# Autodesk Inventor assembly: WheelAssembly3.0
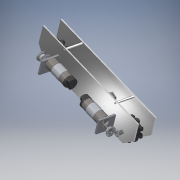
[picture p0: Inventor's stored thumbnail of the model, 180x180]
Saved by Autodesk Inventor 2019 (Build 230136000, 136)
## iProperties
Created: 2017-07-22
Part Number: WheelAssembly3.0
Document SubType Name: Assembly
Designer: User
Mass: 2301.48 g
Surface Area: 4071.67 cm^2
Volume: 902.346 cm^3
Density: 2.55055 g/cm^3
Author: User
## Documents named in this file (23)
- C:\Robotics\CAD\2020-21-CAD\Drivetrain\drive train left.iam
- C:\Robotics\CAD\2016-17_CAD\Custom COTS\4inax.ipt
- C:\Robotics\CAD\COTSParts\Actobotics\535 parts\535198Bearing.25ID.5OD.ipt
- C:\Robotics\CAD\COTSParts\Actobotics\Collar.ipt
- C:\Robotics\CAD\COTSParts\Fasteners\6-32 SHCS x500.ipt
- C:\Robotics\CAD\COTSParts\Fasteners\Hex Standoff 6-32 x2250.ipt
- C:\Robotics\CAD\COTSParts\Motors\am-3102NeveRest20 (1)_MIR.ipt
- C:\Robotics\CAD\COTSParts\Rev\REV-41-1657MecanumWheelRight.iam
- C:\Robotics\CAD\2020-21-CAD\Drivetrain\motor mount.ipt
- C:\Robotics\CAD\COTSParts\Tetrix\Tetrix hub - motor.ipt
- C:\Robotics\CAD\2016-17_CAD\Custom COTS\4inax_MIR1.ipt
- C:\Robotics\CAD\COTSParts\Actobotics\535 parts\535198Bearing.25ID.5OD_MIR1.ipt
- C:\Robotics\CAD\COTSParts\Actobotics\Collar_MIR1.ipt
- C:\Robotics\CAD\COTSParts\Rev\REV-41-1657MecanumWheelRight_MIR.iam
- C:\Robotics\CAD\2020-21-CAD\Drivetrain\motor mount_MIR.ipt
- C:\Robotics\CAD\COTSParts\Motors\am-3102NeveRest20 (1)_MIR_MIR.ipt
- C:\Robotics\CAD\COTSParts\andymark\am-3902 am-3903 2in Omni 14mm Hex.ipt
- C:\Robotics\CAD\COTSParts\Rev\REV-11-1271.STEP encoders.ipt
- C:\Robotics\CAD\COTSParts\Actobotics\637 parts\637222 beval gear\615456 13tooth beval gear.ipt
- C:\Robotics\CAD\COTSParts\Actobotics\637 parts\637222 beval gear\615460 26 tooth beval gear.ipt
- C:\Robotics\CAD\COTSParts\Tetrix\Tetrix Hub - axle.ipt
- C:\Robotics\CAD\2020-21-CAD\Drivetrain\InvertedDrivePlateOutsideright.ipt
- C:\Robotics\CAD\2020-21-CAD\Drivetrain\InvertedDrivePlateInsideleft.ipt
## Components (37 placed, 22 different names)
1. 4inax:4 — Mate:63, Mate:69, Mate:118, Mate:144, Mate:168, Mate:170
2. 535198Bearing.25ID.5OD:1 — Mate:116, Mate:145, Mate:171
3. Collar:1 — Mate:168, Mate:169
4. 535198Bearing.25ID.5OD:5 — Mate:117, Mate:118, Mate:169
5. Hex Standoff 6-32 x2250:1 — Mate:138, Mate:139
6. Hex Standoff 6-32 x2250:2 — Mate:114, Mate:130
7. Hex Standoff 6-32 x2250:3 — Mate:136, Mate:137
8. Hex Standoff 6-32 x2250:4 — Mate:140, Mate:141, Mate:146
9. 6-32 SHCS x500:22 — Mate:119, Mate:149
10. 6-32 SHCS x500:23 — Mate:124, Mate:125, Mate:141
11. 6-32 SHCS x500:24 — Mate:128, Mate:134, Mate:139
12. 6-32 SHCS x500:25 — Mate:129, Mate:130, Mate:131
13. 6-32 SHCS x500:26 — Mate:147, Mate:148
14. 6-32 SHCS x500:27 — Mate:132, Mate:135, Mate:137
15. 6-32 SHCS x500:28 — Mate:154, Mate:157
16. 6-32 SHCS x500:29 — Mate:155, Mate:156
17. REV-41-1657MecanumWheelRight:1 [sub-assembly] — Mate:63, Mate:70, Mate:71, Mate:72, Flush:14
18. motor mount:1 — Mate:66, Mate:67, Mate:113, Flush:16, Flush:20, Mate:162
19. am-3102NeveRest20 (1)_MIR:2 — Mate:66, Mate:67, Mate:112, Angle:8
20. Tetrix hub - motor:1 — Mate:69, Mate:70, Mate:71, Mate:72
21. 4inax_MIR1:1 — Mate:76, Mate:150, Mate:167, Mate:172, Mate:175
22. 535198Bearing.25ID.5OD_MIR1:1 — Mate:151, Mate:174
23. Collar_MIR1:1 — Mate:172, Mate:173
24. 535198Bearing.25ID.5OD_MIR1:2 — Mate:142, Mate:143, Mate:167, Mate:173
25. REV-41-1657MecanumWheelRight_MIR:1 [sub-assembly] — Mate:76, Flush:14, Mate:152
26. motor mount_MIR:1 — Angle:7, Mate:163, Flush:21, Flush:22, Mate:164, Mate:165, Mate:166
27. am-3102NeveRest20 (1)_MIR_MIR:1 — Mate:96, Angle:7, Mate:164, Mate:165, Angle:8
28. am-3902 am-3903 2in Omni 14mm Hex:1 — Mate:89, Mate:90
29. REV-11-1271.STEP encoders:1 — Mate:89, Mate:90, Mate:126, Mate:127, Angle:3
30. 615456 13tooth beval gear:1 — Mate:174, Mate:175
31. 615460 26 tooth beval gear:1 — Mate:93, Mate:94, Mate:96
32. Tetrix Hub - axle:1 — Mate:93, Mate:94, Mate:166
33. 615456 13tooth beval gear:2 — Mate:170, Mate:171
34. 615460 26 tooth beval gear:3 — Mate:113
35. Tetrix Hub - axle:3 — Mate:112
36. InvertedDrivePlateOutsideright:1 — Mate:114, Mate:116, Mate:117, Mate:119, Mate:124, Mate:125, Mate:126, Mate:127, Angle:3, Mate:128, Mate:129, Mate:131, Mate:132, Mate:134, Mate:135, Mate:136, Mate:138, Mate:140, Mate:142, Mate:143, Angle:4, Flush:16, Flush:20
37. InvertedDrivePlateInsideleft:1 — Mate:144, Mate:145, Mate:146, Angle:4, Mate:147, Mate:148, Mate:149, Mate:150, Mate:151, Mate:152, Mate:154, Mate:155, Mate:156, Mate:157, Mate:162, Mate:163, Flush:21, Flush:22
## Relationships (77: Mate 68, Flush 5, Angle 4)
- Mate:63: 4inax:4 ↔ REV-41-1657MecanumWheelRight:1
- Mate:66: motor mount:1 ↔ am-3102NeveRest20 (1)_MIR:2
- Mate:67: motor mount:1 ↔ am-3102NeveRest20 (1)_MIR:2
- Mate:69: 4inax:4 ↔ Tetrix hub - motor:1
- Mate:70: REV-41-1657MecanumWheelRight:1 ↔ Tetrix hub - motor:1
- Mate:71: REV-41-1657MecanumWheelRight:1 ↔ Tetrix hub - motor:1
- Mate:72: REV-41-1657MecanumWheelRight:1 ↔ Tetrix hub - motor:1
- Mate:76: 4inax_MIR1:1 ↔ REV-41-1657MecanumWheelRight_MIR:1
- Flush:14: REV-41-1657MecanumWheelRight:1 ↔ REV-41-1657MecanumWheelRight_MIR:1
- Mate:89: am-3902 am-3903 2in Omni 14mm Hex:1 ↔ REV-11-1271.STEP encoders:1
- Mate:90: am-3902 am-3903 2in Omni 14mm Hex:1 ↔ REV-11-1271.STEP encoders:1
- Mate:93: 615460 26 tooth beval gear:1 ↔ Tetrix Hub - axle:1
- Mate:94: 615460 26 tooth beval gear:1 ↔ Tetrix Hub - axle:1
- Mate:96: am-3102NeveRest20 (1)_MIR_MIR:1 ↔ 615460 26 tooth beval gear:1
- [Mate]: 615460 26 tooth beval gear:3 ↔ Tetrix Hub - axle:3
- [Mate]: 615460 26 tooth beval gear:3 ↔ Tetrix Hub - axle:3
- Mate:112: am-3102NeveRest20 (1)_MIR:2 ↔ Tetrix Hub - axle:3
- Mate:113 (25.4 mm): motor mount:1 ↔ 615460 26 tooth beval gear:3
- Mate:114: Hex Standoff 6-32 x2250:2 ↔ InvertedDrivePlateOutsideright:1
- Mate:116: 535198Bearing.25ID.5OD:1 ↔ InvertedDrivePlateOutsideright:1
- Mate:117: 535198Bearing.25ID.5OD:5 ↔ InvertedDrivePlateOutsideright:1
- Mate:118: 4inax:4 ↔ 535198Bearing.25ID.5OD:5
- Mate:119: 6-32 SHCS x500:22 ↔ InvertedDrivePlateOutsideright:1
- Mate:124: 6-32 SHCS x500:23 ↔ InvertedDrivePlateOutsideright:1
- Mate:125: 6-32 SHCS x500:23 ↔ InvertedDrivePlateOutsideright:1
- Mate:126: REV-11-1271.STEP encoders:1 ↔ InvertedDrivePlateOutsideright:1
- Mate:127: REV-11-1271.STEP encoders:1 ↔ InvertedDrivePlateOutsideright:1
- Angle:3 (25.25 deg): REV-11-1271.STEP encoders:1 ↔ InvertedDrivePlateOutsideright:1
- Mate:128: 6-32 SHCS x500:24 ↔ InvertedDrivePlateOutsideright:1
- Mate:129: 6-32 SHCS x500:25 ↔ InvertedDrivePlateOutsideright:1
- Mate:130: Hex Standoff 6-32 x2250:2 ↔ 6-32 SHCS x500:25
- Mate:131: 6-32 SHCS x500:25 ↔ InvertedDrivePlateOutsideright:1
- Mate:132: 6-32 SHCS x500:27 ↔ InvertedDrivePlateOutsideright:1
- Mate:134: 6-32 SHCS x500:24 ↔ InvertedDrivePlateOutsideright:1
- Mate:135: 6-32 SHCS x500:27 ↔ InvertedDrivePlateOutsideright:1
- Mate:136: Hex Standoff 6-32 x2250:3 ↔ InvertedDrivePlateOutsideright:1
- Mate:137: Hex Standoff 6-32 x2250:3 ↔ 6-32 SHCS x500:27
- Mate:138: Hex Standoff 6-32 x2250:1 ↔ InvertedDrivePlateOutsideright:1
- Mate:139: Hex Standoff 6-32 x2250:1 ↔ 6-32 SHCS x500:24
- Mate:140: Hex Standoff 6-32 x2250:4 ↔ InvertedDrivePlateOutsideright:1
- Mate:141: Hex Standoff 6-32 x2250:4 ↔ 6-32 SHCS x500:23
- Mate:142: 535198Bearing.25ID.5OD_MIR1:2 ↔ InvertedDrivePlateOutsideright:1
- Mate:143: 535198Bearing.25ID.5OD_MIR1:2 ↔ InvertedDrivePlateOutsideright:1
- Mate:144: 4inax:4 ↔ InvertedDrivePlateInsideleft:1
- Mate:145: 535198Bearing.25ID.5OD:1 ↔ InvertedDrivePlateInsideleft:1
- Mate:146: Hex Standoff 6-32 x2250:4 ↔ InvertedDrivePlateInsideleft:1
- Angle:4 (0 deg): InvertedDrivePlateOutsideright:1 ↔ InvertedDrivePlateInsideleft:1
- Mate:147: 6-32 SHCS x500:26 ↔ InvertedDrivePlateInsideleft:1
- Mate:148: 6-32 SHCS x500:26 ↔ InvertedDrivePlateInsideleft:1
- Mate:149: 6-32 SHCS x500:22 ↔ InvertedDrivePlateInsideleft:1
- Mate:150: 4inax_MIR1:1 ↔ InvertedDrivePlateInsideleft:1
- Mate:151: 535198Bearing.25ID.5OD_MIR1:1 ↔ InvertedDrivePlateInsideleft:1
- Mate:152 (25.4 mm): REV-41-1657MecanumWheelRight_MIR:1 ↔ InvertedDrivePlateInsideleft:1
- Mate:154: 6-32 SHCS x500:28 ↔ InvertedDrivePlateInsideleft:1
- Mate:155: 6-32 SHCS x500:29 ↔ InvertedDrivePlateInsideleft:1
- Mate:156: 6-32 SHCS x500:29 ↔ InvertedDrivePlateInsideleft:1
- Mate:157: 6-32 SHCS x500:28 ↔ InvertedDrivePlateInsideleft:1
- Flush:16 (82.55 mm): motor mount:1 ↔ InvertedDrivePlateOutsideright:1
- Angle:7 (17 deg): motor mount_MIR:1 ↔ am-3102NeveRest20 (1)_MIR_MIR:1
- Flush:20 (12.7 mm): motor mount:1 ↔ InvertedDrivePlateOutsideright:1
- Mate:162: motor mount:1 ↔ InvertedDrivePlateInsideleft:1
- Mate:163: motor mount_MIR:1 ↔ InvertedDrivePlateInsideleft:1
- Flush:21 (12.7 mm): motor mount_MIR:1 ↔ InvertedDrivePlateInsideleft:1
- Flush:22 (88.9 mm): motor mount_MIR:1 ↔ InvertedDrivePlateInsideleft:1
- Mate:164: motor mount_MIR:1 ↔ am-3102NeveRest20 (1)_MIR_MIR:1
- Mate:165: motor mount_MIR:1 ↔ am-3102NeveRest20 (1)_MIR_MIR:1
- Mate:166 (25.4 mm): motor mount_MIR:1 ↔ Tetrix Hub - axle:1
- Mate:167: 4inax_MIR1:1 ↔ 535198Bearing.25ID.5OD_MIR1:2
- Mate:168: 4inax:4 ↔ Collar:1
- Mate:169: Collar:1 ↔ 535198Bearing.25ID.5OD:5
- Mate:170: 4inax:4 ↔ 615456 13tooth beval gear:2
- Mate:171 (6.35 mm): 535198Bearing.25ID.5OD:1 ↔ 615456 13tooth beval gear:2
- Mate:172: 4inax_MIR1:1 ↔ Collar_MIR1:1
- Mate:173: Collar_MIR1:1 ↔ 535198Bearing.25ID.5OD_MIR1:2
- Mate:174 (6.35 mm): 535198Bearing.25ID.5OD_MIR1:1 ↔ 615456 13tooth beval gear:1
- Mate:175: 4inax_MIR1:1 ↔ 615456 13tooth beval gear:1
- Angle:8 (0 deg): am-3102NeveRest20 (1)_MIR:2 ↔ am-3102NeveRest20 (1)_MIR_MIR:1
## Named parameters: d382_d360 = 0 mm, d383_d361 = 0 mm
